# Autodesk Inventor assembly: Assembly3
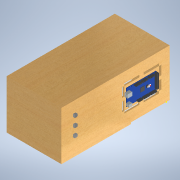
[picture p0: Inventor's stored thumbnail of the model, 180x180]
Saved by Autodesk Inventor 2022.2 (Build 262287000, 287)
## iProperties
Created: 2022-02-28
Part Number: Assembly3
Document SubType Name: Assembly
Designer: PRASHANTH
Author: PRASHANTH
## Documents named in this file (4)
- E:\BME\Autodesk Sample\Engg Exploration\Subsystem3-Button Unit\Assembly3.iam
- E:\BME\Autodesk Sample\Engg Exploration\Subsystem3-Button Unit\button unit.ipt
- E:\BME\Autodesk Sample\Engg Exploration\Subsystem3-Button Unit\Arduino Mega main part.ipt
- E:\BME\Autodesk Sample\Engg Exploration\Subsystem3-Button Unit\Buttons.ipt
## Components (5 placed, 3 different names)
1. button unit:1 — Mate:1, Flush:1, Flush:2, Mate:2, Mate:3, Mate:4
2. Arduino Mega main part:1 — Mate:1, Flush:1, Flush:2
3. Buttons:1 — Mate:2, Flush:3
4. Buttons:2 — Mate:3, Flush:4
5. Buttons:3 — Mate:4, Flush:3, Flush:4
## Relationships (8: Mate 4, Flush 4)
- Mate:1: button unit:1 ↔ Arduino Mega main part:1
- Flush:1 (8 mm): button unit:1 ↔ Arduino Mega main part:1
- Flush:2 (-7 mm): button unit:1 ↔ Arduino Mega main part:1
- Mate:2: button unit:1 ↔ Buttons:1
- Mate:3: button unit:1 ↔ Buttons:2
- Mate:4: button unit:1 ↔ Buttons:3
- Flush:3: Buttons:1 ↔ Buttons:3
- Flush:4: Buttons:2 ↔ Buttons:3
